# Autodesk Inventor assembly: CajaCNC
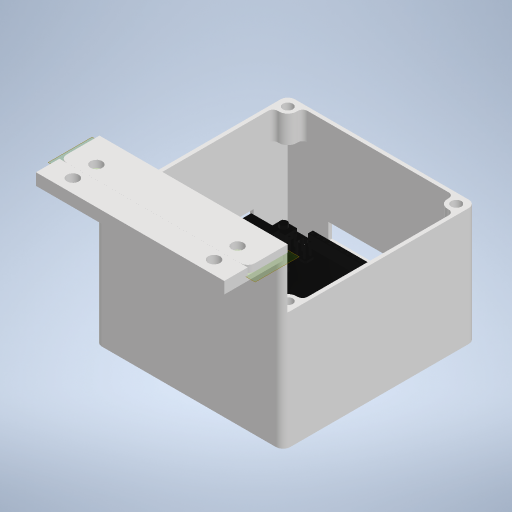
[picture p0: Inventor's stored thumbnail of the model, 512x512]
Saved by Autodesk Inventor 2024 (Build 280153000, 153)
## iProperties
Created: 2023-04-03
Part Number: CajaCNC
Document SubType Name: Assembly
Designer: sergi
Author: sergi
## Documents named in this file (5)
- C:\Users\sergi\OneDrive\Escritorio\proyectos\Objetos 3d\CajaCNC\CajaCNC.iam
- C:\Users\sergi\OneDrive\Escritorio\proyectos\Objetos 3d\Bomba Persitaltica\Ventilador.ipt
- C:\Users\sergi\OneDrive\Escritorio\proyectos\Objetos 3d\Bomba Persitaltica\Caja.ipt
- C:\Users\sergi\Downloads\Imported Components\arduino_uno\arduino_uno.ipt
- C:\Users\sergi\OneDrive\Escritorio\proyectos\Objetos 3d\CajaCNC\Adaptador.ipt
## Components (4 placed, 4 different names)
1. Ventilador:1 — Nivelación:1
2. Caja:1 — Nivelación:1, Coincidencia:1, Coincidencia:3, Coincidencia:4, Nivelación:2, Nivelación:3
3. arduino_uno:1 — Coincidencia:1, Coincidencia:3, Coincidencia:4
4. Adaptador:1 — Nivelación:2, Nivelación:3
## Relationships (6: Flush 3, Mate 3)
- Nivelación:1 [Flush]: Ventilador:1 ↔ Caja:1
- Coincidencia:1 [Mate] (5 mm): Caja:1 ↔ arduino_uno:1
- Coincidencia:3 [Mate]: Caja:1 ↔ arduino_uno:1
- Coincidencia:4 [Mate] (17 mm): Caja:1 ↔ arduino_uno:1
- Nivelación:2 [Flush]: Caja:1 ↔ Adaptador:1
- Nivelación:3 [Flush]: Caja:1 ↔ Adaptador:1
